# Autodesk Inventor assembly: Assembly1
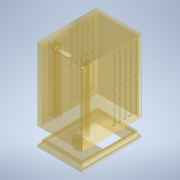
[picture p0: Inventor's stored thumbnail of the model, 180x180]
Saved by Autodesk Inventor 2022 (Build 260153000, 153)
## iProperties
Created: 2022-01-12
Part Number: Assembly1
Document SubType Name: Assembly
Designer: chad
Author: chad
## Documents named in this file (3)
- F:\Documents\eCO2 Monitor\Enclosure\Enclosure v2.iam
- F:\Documents\eCO2 Monitor\Enclosure\Front.ipt
- F:\Documents\eCO2 Monitor\Enclosure\Back.ipt
## Components (2 placed, 2 different names)
1. Front:1 — Mate:1, Flush:1
2. Back:1 — Mate:1, Flush:1
## Relationships (2: Mate 1, Flush 1)
- Mate:1 (15 mm): Front:1 ↔ Back:1
- Flush:1: Front:1 ↔ Back:1
